# Autodesk Inventor assembly: base4kaki
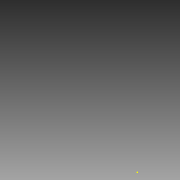
[picture p0: Inventor's stored thumbnail of the model, 180x180]
Saved by Autodesk Inventor 2015 (Build 190159000, 159)
## iProperties
Created: 2015-01-15
Part Number: base4kaki
Document SubType Name: Assembly
Designer: Rafi Kurnia Putra
Author: Rafi Kurnia Putra
## Documents named in this file (8)
- D:\Dropbox\krpai berkaki trui 2015\ROBUSTA\MEKANIK\Grand design\base\base4kaki.iam
- D:\Dropbox\krpai berkaki trui 2015\ROBUSTA\MEKANIK\Grand design\base\BAWAH4.ipt
- D:\Dropbox\krpai berkaki trui 2015\ROBUSTA\MEKANIK\Grand design\base\ATAS4baru.ipt
- D:\Dropbox\krpai berkaki trui 2015\ROBUSTA\MEKANIK\Grand design\base\bawahdepan.ipt
- D:\Dropbox\krpai berkaki trui 2015\ROBUSTA\MEKANIK\Grand design\base\spacer 5 cm.ipt
- D:\Dropbox\krpai berkaki trui 2015\ROBUSTA\MEKANIK\Grand design\base\bawahbelakangbaru.ipt
- D:\Dropbox\krpai berkaki trui 2015\ROBUSTA\MEKANIK\Grand design\base\spacer 1 cm.ipt
- D:\Downloads\Compressed\servohorns.sldwks\Imported Components\HMSH-01\HMSH-01.ipt
## Components (13 placed, 7 different names)
1. BAWAH4:1 — Mate:10, Mate:11, Mate:12, Mate:19, Mate:20, Mate:21, Insert:9, Insert:10, Mate:28, Mate:29, Mate:30
2. ATAS4baru:1 — Insert:1, Insert:2, Insert:3, Insert:4, Insert:5, Insert:6, Insert:7, Insert:8, Mate:31
3. bawahdepan:1 — Mate:10, Mate:11, Mate:12
4. bawahbelakangbaru:1 — Mate:19, Mate:20, Mate:21, Mate:28, Mate:29, Mate:30
5. spacer 1 cm:1 — Insert:1
6. spacer 1 cm:2 — Insert:4
7. spacer 1 cm:3 — Insert:3
8. spacer 1 cm:4 — Insert:2
9. spacer 5 cm:1 — Insert:5, Insert:10
10. spacer 5 cm:2 — Insert:7
11. spacer 5 cm:3 — Insert:8
12. spacer 5 cm:4 — Insert:6, Insert:9
13. HMSH-01:1 — Mate:31
## Relationships (20: Mate 10, Insert 10)
- Mate:10: BAWAH4:1 ↔ bawahdepan:1
- Mate:11: BAWAH4:1 ↔ bawahdepan:1
- Mate:12: BAWAH4:1 ↔ bawahdepan:1
- Mate:19: BAWAH4:1 ↔ bawahbelakangbaru:1
- Mate:20: BAWAH4:1 ↔ bawahbelakangbaru:1
- Mate:21: BAWAH4:1 ↔ bawahbelakangbaru:1
- Insert:1: ATAS4baru:1 ↔ spacer 1 cm:1
- Insert:2: ATAS4baru:1 ↔ spacer 1 cm:4
- Insert:3: ATAS4baru:1 ↔ spacer 1 cm:3
- Insert:4: ATAS4baru:1 ↔ spacer 1 cm:2
- Insert:5: ATAS4baru:1 ↔ spacer 5 cm:1
- Insert:6: ATAS4baru:1 ↔ spacer 5 cm:4
- Insert:7: ATAS4baru:1 ↔ spacer 5 cm:2
- Insert:8: ATAS4baru:1 ↔ spacer 5 cm:3
- Insert:9: BAWAH4:1 ↔ spacer 5 cm:4
- Insert:10: BAWAH4:1 ↔ spacer 5 cm:1
- Mate:28: BAWAH4:1 ↔ bawahbelakangbaru:1
- Mate:29: BAWAH4:1 ↔ bawahbelakangbaru:1
- Mate:30: BAWAH4:1 ↔ bawahbelakangbaru:1
- Mate:31: ATAS4baru:1 ↔ HMSH-01:1
